# Autodesk Inventor assembly: Столб_переда_корпуса_2.0
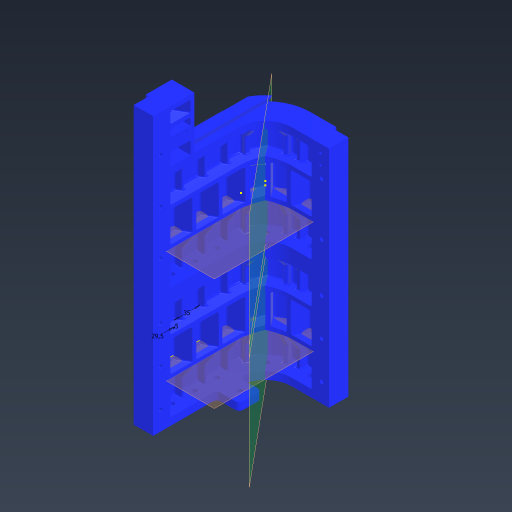
[picture p0: Inventor's stored thumbnail of the model, 512x512]
Saved by Autodesk Inventor 2023.2 (Build 272271030, 271C)
## iProperties
Created: 2025-10-02
Part Number: Столб_переда_корпуса_2.0
Document SubType Name: Assembly
Designer: Олег Коноваленко
Author: Олег Коноваленко
## Documents named in this file (3)
- D:\!Rover\Rover\Rover_construction\Столб_переда_корпуса_2.0.iam
- D:\!Rover\Rover\Rover_construction\Столб_версия_2.0.ipt
- D:\!Rover\Rover\Rover_construction\2.0_столб_переда.ipt
## Components (2 placed, 2 different names)
1. Столб_версия_2.0:1 — Совмещение:1, Заподлицо:1, Заподлицо:2
2. 2.0_столб_переда:1 — Совмещение:1, Заподлицо:1, Заподлицо:2
## Relationships (3: Flush 2, Mate 1)
- Совмещение:1 [Mate]: Столб_версия_2.0:1 ↔ 2.0_столб_переда:1
- Заподлицо:1 [Flush]: Столб_версия_2.0:1 ↔ 2.0_столб_переда:1
- Заподлицо:2 [Flush]: Столб_версия_2.0:1 ↔ 2.0_столб_переда:1
